# Autodesk Inventor assembly: Omniscope_new_v0
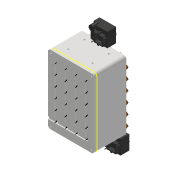
[picture p0: Inventor's stored thumbnail of the model, 180x180]
Saved by Autodesk Inventor 2022 (Build 260153000, 153)
## iProperties
Created: 2022-05-25
Part Number: Omniscope_new_v0
Document SubType Name: Assembly
Designer: diederichbenedict
Author: diederichbenedict
## Documents named in this file (9)
- C:\Users\diederichbenedict\Dropbox\Dokumente\Promotion\PROJECTS\Omniscope\INVENTOR\Omniscope_new_v0.iam
- C:\Users\diederichbenedict\Dropbox\Dokumente\Promotion\PROJECTS\Omniscope\INVENTOR\00_MicroSDCard.ipt
- C:\Users\diederichbenedict\Dropbox\Dokumente\Promotion\PROJECTS\Omniscope\INVENTOR\Omniscope_Base_v0.ipt
- C:\Users\diederichbenedict\Dropbox\Dokumente\Promotion\PROJECTS\Omniscope\INVENTOR\Omniscope_sidewalls_v0.ipt
- C:\Users\diederichbenedict\Dropbox\Dokumente\Promotion\PROJECTS\Omniscope\INVENTOR\OV_Camera.ipt
- C:\Users\diederichbenedict\Dropbox\Dokumente\Promotion\PROJECTS\Omniscope\INVENTOR\00_ESP3-CAMboard.iam
- C:\Users\diederichbenedict\Dropbox\Dokumente\Promotion\PROJECTS\Omniscope\INVENTOR\Omniscope_Camera_fix.ipt
- C:\Users\diederichbenedict\Dropbox\Dokumente\Promotion\PROJECTS\Omniscope\INVENTOR\00_24wellplate_base.ipt
- C:\Users\diederichbenedict\Dropbox\Dokumente\Promotion\PROJECTS\Omniscope\INVENTOR\00_Z_Focus_CCTV_Camera.ipt
## Components (102 placed, 8 different names)
1. Omniscope_Base_v0:1 — Passend:1, Passend:2, Passend:3, Fluchtend:3, Fluchtend:4
2. Omniscope_sidewalls_v0:1 — Fluchtend:3, Fluchtend:4, Passend:7, Fluchtend:7, Fluchtend:15, Fluchtend:16, Passend:8, Passend:9, Passend:10, Fluchtend:17
3. 00_24wellplate_base:1 — Passend:7, Fluchtend:7
4. 00_Z_Focus_CCTV_Camera:1 — Fluchtend:13, Fluchtend:14, Fluchtend:15, Passend:9
5. 00_Z_Focus_CCTV_Camera:2 — Fluchtend:14, Fluchtend:16, Passend:8
6. 00_Z_Focus_CCTV_Camera:3 — Fluchtend:13, Passend:10, Fluchtend:17
7. 00_MicroSDCard:1 — Passend:1, Passend:2, Fluchtend:1, Fluchtend:2
8. 00_ESP3-CAMboard:1 — Fluchtend:1, Fluchtend:2, Passend:3
9. 00_MicroSDCard:2
10. 00_ESP3-CAMboard:2
11. 00_MicroSDCard:3
12. 00_ESP3-CAMboard:3
13. 00_MicroSDCard:4
14. 00_ESP3-CAMboard:4
15. 00_MicroSDCard:5
16. 00_ESP3-CAMboard:5
17. 00_MicroSDCard:6
18. 00_ESP3-CAMboard:6
19. 00_MicroSDCard:7
20. 00_ESP3-CAMboard:7
21. 00_MicroSDCard:8
22. 00_ESP3-CAMboard:8
23. 00_MicroSDCard:9
24. 00_ESP3-CAMboard:9
25. 00_MicroSDCard:10
26. 00_ESP3-CAMboard:10
27. 00_MicroSDCard:11
28. 00_ESP3-CAMboard:11
29. 00_MicroSDCard:12
30. 00_ESP3-CAMboard:12
31. 00_MicroSDCard:13
32. 00_ESP3-CAMboard:13
33. 00_MicroSDCard:14
34. 00_ESP3-CAMboard:14
35. 00_MicroSDCard:15
36. 00_ESP3-CAMboard:15
37. 00_MicroSDCard:16
38. 00_ESP3-CAMboard:16
39. 00_MicroSDCard:17
40. 00_ESP3-CAMboard:17
41. 00_MicroSDCard:18
42. 00_ESP3-CAMboard:18
43. 00_MicroSDCard:19
44. 00_ESP3-CAMboard:19
45. 00_MicroSDCard:20
46. 00_ESP3-CAMboard:20
47. 00_MicroSDCard:21
48. 00_ESP3-CAMboard:21
49. 00_MicroSDCard:22
50. 00_ESP3-CAMboard:22
51. 00_MicroSDCard:23
52. 00_ESP3-CAMboard:23
53. 00_MicroSDCard:24
54. 00_ESP3-CAMboard:24
55. Omniscope_Camera_fix:1
56. OV_Camera:1
57. Omniscope_Camera_fix:2
58. OV_Camera:2
59. Omniscope_Camera_fix:3
60. OV_Camera:3
61. Omniscope_Camera_fix:4
62. OV_Camera:4
63. Omniscope_Camera_fix:5
64. OV_Camera:5
65. Omniscope_Camera_fix:6
66. OV_Camera:6
67. Omniscope_Camera_fix:7
68. OV_Camera:7
69. Omniscope_Camera_fix:8
70. OV_Camera:8
71. Omniscope_Camera_fix:9
72. OV_Camera:9
73. Omniscope_Camera_fix:10
74. OV_Camera:10
75. Omniscope_Camera_fix:11
76. OV_Camera:11
77. Omniscope_Camera_fix:12
78. OV_Camera:12
79. Omniscope_Camera_fix:13
80. OV_Camera:13
81. Omniscope_Camera_fix:14
82. OV_Camera:14
83. Omniscope_Camera_fix:15
84. OV_Camera:15
85. Omniscope_Camera_fix:16
86. OV_Camera:16
87. Omniscope_Camera_fix:17
88. OV_Camera:17
89. Omniscope_Camera_fix:18
90. OV_Camera:18
91. Omniscope_Camera_fix:19
92. OV_Camera:19
93. Omniscope_Camera_fix:20
94. OV_Camera:20
95. Omniscope_Camera_fix:21
96. OV_Camera:21
97. Omniscope_Camera_fix:22
98. OV_Camera:22
99. Omniscope_Camera_fix:23
100. OV_Camera:23
101. Omniscope_Camera_fix:24
102. OV_Camera:24
## Component patterns: (24 elements, first: 00_MicroSDCard:1 + 00_ESP3-CAMboard:1), (24 elements, first: Omniscope_Camera_fix:1 + OV_Camera:1)
## Relationships (17: Flush 10, Mate 7)
- Passend:1 [Mate]: Omniscope_Base_v0:1 ↔ 00_MicroSDCard:1
- Passend:2 [Mate]: Omniscope_Base_v0:1 ↔ 00_MicroSDCard:1
- Fluchtend:1 [Flush]: 00_MicroSDCard:1 ↔ 00_ESP3-CAMboard:1
- Fluchtend:2 [Flush]: 00_MicroSDCard:1 ↔ 00_ESP3-CAMboard:1
- Passend:3 [Mate] (14 mm): Omniscope_Base_v0:1 ↔ 00_ESP3-CAMboard:1
- Fluchtend:3 [Flush]: Omniscope_Base_v0:1 ↔ Omniscope_sidewalls_v0:1
- Fluchtend:4 [Flush]: Omniscope_Base_v0:1 ↔ Omniscope_sidewalls_v0:1
- Passend:7 [Mate]: Omniscope_sidewalls_v0:1 ↔ 00_24wellplate_base:1
- Fluchtend:7 [Flush]: Omniscope_sidewalls_v0:1 ↔ 00_24wellplate_base:1
- Fluchtend:13 [Flush]: 00_Z_Focus_CCTV_Camera:1 ↔ 00_Z_Focus_CCTV_Camera:3
- Fluchtend:14 [Flush]: 00_Z_Focus_CCTV_Camera:1 ↔ 00_Z_Focus_CCTV_Camera:2
- Fluchtend:15 [Flush] (3 mm): Omniscope_sidewalls_v0:1 ↔ 00_Z_Focus_CCTV_Camera:1
- Fluchtend:16 [Flush] (3 mm): Omniscope_sidewalls_v0:1 ↔ 00_Z_Focus_CCTV_Camera:2
- Passend:8 [Mate] (3 mm): Omniscope_sidewalls_v0:1 ↔ 00_Z_Focus_CCTV_Camera:2
- Passend:9 [Mate] (3 mm): Omniscope_sidewalls_v0:1 ↔ 00_Z_Focus_CCTV_Camera:1
- Passend:10 [Mate] (3 mm): Omniscope_sidewalls_v0:1 ↔ 00_Z_Focus_CCTV_Camera:3
- Fluchtend:17 [Flush]: Omniscope_sidewalls_v0:1 ↔ 00_Z_Focus_CCTV_Camera:3
